# Autodesk Inventor assembly: CombineTestRig
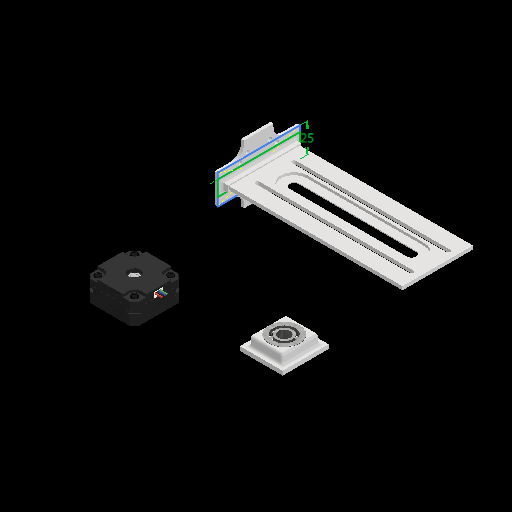
[picture p0: Inventor's stored thumbnail of the model, 512x512]
Saved by Autodesk Inventor 2025 (Build 290162000, 162)
## iProperties
Created: 2025-01-20
Part Number: CombineTestRig
Document SubType Name: Assembly
Designer: Trevor
Author: Trevor
## Documents named in this file (6)
- C:\Users\Trevor\Documents\GitHub\USA-Robotic-Club-2024\assests\CombineTestRig.iam
- C:\Users\Trevor\Documents\GitHub\USA-Robotic-Club-2024\assests\17hm08-1204s-nema17-pancake-21mm-1.snapshot.2\17HM08-1204S Nema17 Pancake 21mm\17HM08-1204S Nema17 Pancake 21mm.ipt
- C:\Users\Trevor\Documents\GitHub\USA-Robotic-Club-2024\assests\CombineTestHorizontal.ipt
- C:\Users\Trevor\Documents\GitHub\USA-Robotic-Club-2024\assests\CombineTestBase.ipt
- C:\Users\Trevor\Documents\GitHub\USA-Robotic-Club-2024\assests\bearing-10mm-2.snapshot.2\PMG(Si)\PMG(Si).ipt
- C:\Users\Trevor\Documents\GitHub\USA-Robotic-Club-2024\assests\BearingTestMount.ipt
## Components (5 placed, 5 different names)
1. 17HM08-1204S Nema17 Pancake 21mm:1
2. CombineTestHorizontal:1 — Flush:2
3. CombineTestBase:1 — Flush:2
4. PMG(Si):1 — Flush:3
5. BearingTestMount:1 — Flush:3
## Relationships (2: Flush 2)
- Flush:2: CombineTestHorizontal:1 ↔ CombineTestBase:1
- Flush:3: PMG(Si):1 ↔ BearingTestMount:1
